# Autodesk Inventor assembly: Почти готово
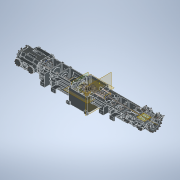
[picture p0: Inventor's stored thumbnail of the model, 180x180]
Saved by Autodesk Inventor 2021 (Build 250183000, 183)
## iProperties
Created: 2020-12-08
Part Number: Почти готово
Document SubType Name: Assembly
Designer: Тимоха
Author: Тимоха
## Documents named in this file (41)
- C:\Users\Тимоха\Desktop\КР Компрессор\compressor\Почти готово.iam
- C:\Users\Тимоха\Desktop\КР Компрессор\compressor\Картер.ipt
- C:\Users\Тимоха\Documents\Inventor\Content Center Files\R2021\ru-RU\Nut GOST 15524-70\Гайка M24-6H ГОСТ 15524-70.ipt
- C:\Users\Тимоха\Documents\Inventor\Content Center Files\R2021\ru-RU\GOST 11371-78  A\Шайба 27 ГОСТ 11371-78.ipt
- C:\Users\Тимоха\Desktop\КР Компрессор\compressor\Почти готово_CPY.iam
- C:\Users\Тимоха\Desktop\КР Компрессор\compressor\Вал.ipt
- C:\Users\Тимоха\Desktop\КР Компрессор\compressor\Нижняя часть коренного подшипника.ipt
- C:\Users\Тимоха\Desktop\КР Компрессор\compressor\Крышка коренного подшипника1.ipt
- C:\Users\Тимоха\Documents\Inventor\Content Center Files\R2021\ru-RU\Stud GOST 22038-76\Шпилька M24-6g×110 ГОСТ 22038-76.ipt
- C:\Users\Тимоха\Desktop\КР Компрессор\compressor\Под шатун.ipt
- C:\Users\Тимоха\Desktop\КР Компрессор\compressor\Шатун.ipt
- C:\Users\Тимоха\Desktop\КР Компрессор\compressor\Крышка стенки картера верх.ipt
- C:\Users\Тимоха\Desktop\КР Компрессор\compressor\Крышка стенки картера низ.ipt
- C:\Users\Тимоха\Desktop\КР Компрессор\compressor\Балка.ipt
- C:\Users\Тимоха\Documents\Inventor\Content Center Files\R2021\ru-RU\Bolt GOST R 50274-92\Болт M8-6g×16-F ГОСТ Р 50274-92.ipt
- C:\Users\Тимоха\Documents\Inventor\Content Center Files\R2021\ru-RU\Bolt GOST R 50274-92\Болт M8-6g×20-F ГОСТ Р 50274-92.ipt
- C:\Users\Тимоха\Desktop\КР Компрессор\compressor\Крышка картера 1.ipt
- C:\Users\Тимоха\Desktop\КР Компрессор\compressor\Крышка картера 2.ipt
- C:\Users\Тимоха\Desktop\КР Компрессор\compressor\Крышка картера 3.ipt
- C:\Users\Тимоха\Desktop\КР Компрессор\compressor\Крышка картера 4.ipt
- C:\Users\Тимоха\Desktop\КР Компрессор\compressor\Стяжка.ipt
- C:\Users\Тимоха\Documents\Inventor\Content Center Files\R2021\ru-RU\Nut GOST ISO 4034-2014\ГайкаM14ГОСТ ISO 4034-2014.ipt
- C:\Users\Тимоха\Desktop\КР Компрессор\compressor\Под стяжку.ipt
- C:\Users\Тимоха\Desktop\КР Компрессор\compressor\Под стяжку_MIR.ipt
- C:\Users\Тимоха\Desktop\КР Компрессор\compressor\Стяжка_MIR.ipt
- C:\Users\Тимоха\Desktop\КР Компрессор\compressor\Под стяжку_MIR1.ipt
- C:\Users\Тимоха\Desktop\КР Компрессор\compressor\Под стяжку_MIR_MIR.ipt
- C:\Users\Тимоха\Desktop\КР Компрессор\compressor\Корпус дросселя.ipt
- C:\Users\Тимоха\Desktop\КР Компрессор\compressor\Корпус сальника 1.ipt
- C:\Users\Тимоха\Desktop\КР Компрессор\compressor\Корпус сальника 2.ipt
- C:\Users\Тимоха\Desktop\КР Компрессор\compressor\Корпус сальника 3.ipt
- C:\Users\Тимоха\Desktop\КР Компрессор\compressor\Корпус сальника 4.ipt
- C:\Users\Тимоха\Desktop\КР Компрессор\compressor\Корпус сальника0.ipt
- C:\Users\Тимоха\Desktop\КР Компрессор\compressor\Крышка сальников.ipt
- C:\Users\Тимоха\Desktop\КР Компрессор\compressor\В сальник.ipt
- C:\Users\Тимоха\Desktop\КР Компрессор\compressor\Дроссельное кольцо.ipt
- C:\Users\Тимоха\Desktop\КР Компрессор\compressor\Кольцо сальника 1.ipt
- C:\Users\Тимоха\Desktop\КР Компрессор\compressor\Кольцо сальника 2.ipt
- C:\Users\Тимоха\Desktop\КР Компрессор\compressor\Кольцо сальника.ipt
- C:\Users\Тимоха\Desktop\КР Компрессор\compressor\Пружина дросселя.ipt
- C:\Users\Тимоха\Desktop\КР Компрессор\compressor\Пружина сальника.ipt
## Components (186 placed, 40 different names)
1. Картер:1 — Жесткий:406, Жесткий:407, Жесткий:410, Жесткий:411, Жесткий:412, Жесткий:421, Жесткий:422, Жесткий:423, Жесткий:428, Жесткий:429, Жесткий:431, Жесткий:433, Жесткий:434, Заподлицо:1, Заподлицо:2, Заподлицо:3, Заподлицо:4, Заподлицо:5, Заподлицо:6, Заподлицо:7, Заподлицо:8, Заподлицо:9, Жесткий:483, Жесткий:484, Заподлицо:14, Заподлицо:15, Заподлицо:16
2. Вал:1 — Цилиндрический:3, Жесткий:426, Совмещение:1, Жесткий:430, С поворотом:4
3. Нижняя часть коренного подшипника:1 — Жесткий:406, Цилиндрический:3, Жесткий:408
4. Нижняя часть коренного подшипника:2 — Жесткий:407, Жесткий:409
5. Нижняя часть коренного подшипника:3 — Жесткий:409
6. Нижняя часть коренного подшипника:4 — Жесткий:408
7. Крышка коренного подшипника1:1 — Жесткий:410
8. Крышка коренного подшипника1:2 — Жесткий:411, Совмещение:1
9. Шпилька ГОСТ 22038-76 M24-6g×110:1 — Жесткий:412, Жесткий:413, Жесткий:414
10. Гайка ГОСТ 15524-70 M24:54 — Жесткий:414
11. Шайба  ГОСТ 11371-78 28:22 — Жесткий:413
12. Шпилька ГОСТ 22038-76 M24-6g×110:2 — Жесткий:421
13. Гайка ГОСТ 15524-70 M24:55
14. Шайба  ГОСТ 11371-78 28:23
15. Шпилька ГОСТ 22038-76 M24-6g×110:3 — Жесткий:423
16. Гайка ГОСТ 15524-70 M24:56
17. Шайба  ГОСТ 11371-78 28:24
18. Шпилька ГОСТ 22038-76 M24-6g×110:4 — Жесткий:422
19. Гайка ГОСТ 15524-70 M24:57
20. Шайба  ГОСТ 11371-78 28:25
21. Под шатун:1 — Жесткий:425
22. Под шатун:2 — Жесткий:425, Жесткий:430
23. Под шатун:3 — Жесткий:426, Жесткий:427
24. Под шатун:4 — Жесткий:427, Цилиндрический:5
25. Почти готово_CPY:1 [sub-assembly] — Жесткий:429, С поворотом:5
26. Почти готово_CPY:2 [sub-assembly] — Жесткий:428, С поворотом:2, Заподлицо:7, Жесткий:546
27. Шатун:2 — Цилиндрический:5, С поворотом:2
28. Крышка стенки картера верх:1 — Жесткий:432, Жесткий:435, Жесткий:436, Жесткий:437, Жесткий:438, Жесткий:439, Жесткий:440, Жесткий:442, Жесткий:443, Жесткий:444, Жесткий:445, Жесткий:446, Жесткий:452, Жесткий:453, Жесткий:454, Жесткий:455, Жесткий:456, Жесткий:457, Жесткий:458
29. Крышка стенки картера низ:1 — Жесткий:431, Жесткий:432, Жесткий:447, Жесткий:448, Жесткий:449, Жесткий:450, Жесткий:451
30. Балка:1 — Жесткий:433
31. Балка:2 — Жесткий:434
32. Болт ГОСТ Р 50274-92 M8-6g×20-F:1 — Жесткий:435
33. Болт ГОСТ Р 50274-92 M8-6g×16-F:1 — Жесткий:439
34. Болт ГОСТ Р 50274-92 M8-6g×16-F:2 — Жесткий:436
35. Болт ГОСТ Р 50274-92 M8-6g×16-F:3 — Жесткий:440
36. Болт ГОСТ Р 50274-92 M8-6g×16-F:5 — Жесткий:438
37. Болт ГОСТ Р 50274-92 M8-6g×16-F:6 — Жесткий:442
38. Болт ГОСТ Р 50274-92 M8-6g×16-F:7 — Жесткий:437
39. Болт ГОСТ Р 50274-92 M8-6g×20-F:2 — Жесткий:443
40. Болт ГОСТ Р 50274-92 M8-6g×16-F:8 — Жесткий:446
41. Болт ГОСТ Р 50274-92 M8-6g×16-F:9 — Жесткий:444
42. Болт ГОСТ Р 50274-92 M8-6g×16-F:10 — Жесткий:450
43. Болт ГОСТ Р 50274-92 M8-6g×16-F:11 — Жесткий:451
44. Болт ГОСТ Р 50274-92 M8-6g×16-F:12 — Жесткий:445
45. Болт ГОСТ Р 50274-92 M8-6g×16-F:13 — Жесткий:447
46. Болт ГОСТ Р 50274-92 M8-6g×16-F:14 — Жесткий:449
47. Болт ГОСТ Р 50274-92 M8-6g×20-F:3 — Жесткий:452
48. Болт ГОСТ Р 50274-92 M8-6g×16-F:19 — Жесткий:448
49. Крышка картера 1:1 — Заподлицо:1, Заподлицо:2, Жесткий:459, Жесткий:460, Жесткий:461, Заподлицо:10, Жесткий:470, Жесткий:471, Жесткий:472, Жесткий:473, Жесткий:474, Жесткий:475, Жесткий:476
50. Крышка картера 2:1 — Заподлицо:3, Заподлицо:4, Жесткий:462, Жесткий:463, Жесткий:464, С поворотом:3, Жесткий:465, Жесткий:466, Жесткий:467, Заподлицо:11, Заподлицо:12
51. Крышка картера 3:1 — Заподлицо:5, Заподлицо:6, Жесткий:468, Жесткий:469, Заподлицо:13
52. Крышка картера 4:1 — Заподлицо:8, Заподлицо:9, Жесткий:477, Жесткий:478, Жесткий:479, Жесткий:480, Жесткий:481, Жесткий:482
53. Болт ГОСТ Р 50274-92 M8-6g×20-F:4 — Жесткий:453
54. Болт ГОСТ Р 50274-92 M8-6g×20-F:12 — Жесткий:471
55. Болт ГОСТ Р 50274-92 M8-6g×20-F:13 — Жесткий:473
56. Болт ГОСТ Р 50274-92 M8-6g×20-F:19 — Жесткий:468
57. Болт ГОСТ Р 50274-92 M8-6g×20-F:20 — Жесткий:469
58. Болт ГОСТ Р 50274-92 M8-6g×20-F:21 — Жесткий:460
59. Болт ГОСТ Р 50274-92 M8-6g×20-F:26 — Жесткий:454
60. Болт ГОСТ Р 50274-92 M8-6g×20-F:27 — Жесткий:463
61. Болт ГОСТ Р 50274-92 M8-6g×20-F:28 — Жесткий:462
62. Болт ГОСТ Р 50274-92 M8-6g×20-F:29 — Жесткий:458
63. Болт ГОСТ Р 50274-92 M8-6g×20-F:30 — Жесткий:465
64. Болт ГОСТ Р 50274-92 M8-6g×20-F:31 — Жесткий:466
65. Болт ГОСТ Р 50274-92 M8-6g×20-F:32 — Жесткий:467
66. Болт ГОСТ Р 50274-92 M8-6g×20-F:33 — Жесткий:455
67. Болт ГОСТ Р 50274-92 M8-6g×20-F:34 — Жесткий:456
68. Болт ГОСТ Р 50274-92 M8-6g×20-F:35 — Жесткий:457
69. Болт ГОСТ Р 50274-92 M8-6g×20-F:36 — Жесткий:461
70. Болт ГОСТ Р 50274-92 M8-6g×20-F:37 — Жесткий:459
71. Болт ГОСТ Р 50274-92 M8-6g×20-F:38 — Жесткий:464
72. Болт ГОСТ Р 50274-92 M8-6g×20-F:39 — С поворотом:3
73. Болт ГОСТ Р 50274-92 M8-6g×20-F:40 — Жесткий:470
74. Болт ГОСТ Р 50274-92 M8-6g×20-F:41 — Жесткий:472
75. Болт ГОСТ Р 50274-92 M8-6g×20-F:42 — Жесткий:474
76. Болт ГОСТ Р 50274-92 M8-6g×20-F:43 — Жесткий:475
77. Болт ГОСТ Р 50274-92 M8-6g×20-F:45 — Жесткий:476
78. Болт ГОСТ Р 50274-92 M8-6g×20-F:47
79. Болт ГОСТ Р 50274-92 M8-6g×20-F:48
80. Болт ГОСТ Р 50274-92 M8-6g×20-F:49
81. Болт ГОСТ Р 50274-92 M8-6g×20-F:50
82. Болт ГОСТ Р 50274-92 M8-6g×20-F:51
83. Болт ГОСТ Р 50274-92 M8-6g×20-F:52
84. Болт ГОСТ Р 50274-92 M8-6g×20-F:53
85. Болт ГОСТ Р 50274-92 M8-6g×20-F:54
86. Болт ГОСТ Р 50274-92 M8-6g×20-F:55
87. Болт ГОСТ Р 50274-92 M8-6g×20-F:56
88. Болт ГОСТ Р 50274-92 M8-6g×20-F:57
89. Болт ГОСТ Р 50274-92 M8-6g×20-F:58
90. Болт ГОСТ Р 50274-92 M8-6g×20-F:59
91. Болт ГОСТ Р 50274-92 M8-6g×20-F:60
92. Болт ГОСТ Р 50274-92 M8-6g×20-F:61
93. Болт ГОСТ Р 50274-92 M8-6g×20-F:62
94. Болт ГОСТ Р 50274-92 M8-6g×20-F:63
95. Болт ГОСТ Р 50274-92 M8-6g×20-F:64
96. Болт ГОСТ Р 50274-92 M8-6g×20-F:65
97. Болт ГОСТ Р 50274-92 M8-6g×20-F:66
98. Болт ГОСТ Р 50274-92 M8-6g×20-F:67
99. Болт ГОСТ Р 50274-92 M8-6g×20-F:68
100. Болт ГОСТ Р 50274-92 M8-6g×20-F:69
101. Болт ГОСТ Р 50274-92 M8-6g×20-F:70
102. Болт ГОСТ Р 50274-92 M8-6g×20-F:71
103. Болт ГОСТ Р 50274-92 M8-6g×20-F:72
104. Болт ГОСТ Р 50274-92 M8-6g×20-F:73
105. Болт ГОСТ Р 50274-92 M8-6g×20-F:74
106. Болт ГОСТ Р 50274-92 M8-6g×20-F:75
107. Болт ГОСТ Р 50274-92 M8-6g×20-F:76
108. Болт ГОСТ Р 50274-92 M8-6g×20-F:77
109. Болт ГОСТ Р 50274-92 M8-6g×20-F:78
110. Болт ГОСТ Р 50274-92 M8-6g×20-F:79
111. Болт ГОСТ Р 50274-92 M8-6g×20-F:80
112. Болт ГОСТ Р 50274-92 M8-6g×20-F:81
113. Болт ГОСТ Р 50274-92 M8-6g×20-F:82
114. Болт ГОСТ Р 50274-92 M8-6g×20-F:83
115. Болт ГОСТ Р 50274-92 M8-6g×20-F:84
116. Болт ГОСТ Р 50274-92 M8-6g×20-F:85
117. Болт ГОСТ Р 50274-92 M8-6g×20-F:86
118. Болт ГОСТ Р 50274-92 M8-6g×20-F:87 — Жесткий:477
119. Болт ГОСТ Р 50274-92 M8-6g×20-F:88 — Жесткий:478
120. Болт ГОСТ Р 50274-92 M8-6g×20-F:89 — Жесткий:480
121. Болт ГОСТ Р 50274-92 M8-6g×20-F:90 — Жесткий:481
122. Болт ГОСТ Р 50274-92 M8-6g×20-F:91 — Жесткий:479
123. Болт ГОСТ Р 50274-92 M8-6g×20-F:92 — Жесткий:482
124. Стяжка:1 — Жесткий:483
125. Гайка ГОСТ ISO 4034-2014 (M14):1 — Жесткий:485
126. Стяжка:2 — Жесткий:484
127. Под стяжку:1 — Заподлицо:14, Заподлицо:15, Жесткий:485, Жесткий:486
128. Гайка ГОСТ ISO 4034-2014 (M14):2 — Жесткий:486
129. Гайка ГОСТ ISO 4034-2014 (M14):3 — Жесткий:487
130. Под стяжку_MIR:1 — Жесткий:487, Жесткий:488
131. Гайка ГОСТ ISO 4034-2014 (M14):4 — Жесткий:488
132. Стяжка_MIR:1
133. Гайка ГОСТ ISO 4034-2014 (M14):5 — Жесткий:489
134. Стяжка_MIR:2
135. Под стяжку_MIR1:1 — Жесткий:489, Жесткий:490
136. Гайка ГОСТ ISO 4034-2014 (M14):6 — Жесткий:490
137. Гайка ГОСТ ISO 4034-2014 (M14):7 — Жесткий:491
138. Под стяжку_MIR_MIR:1 — Жесткий:491, Жесткий:492
139. Гайка ГОСТ ISO 4034-2014 (M14):8 — Жесткий:492
140. Шатун:3 — С поворотом:4, С поворотом:5
141. Корпус дросселя:2
142. Корпус сальника 1:2
143. Корпус сальника 2:2
144. Корпус сальника 3:2
145. Корпус сальника 4:2
146. Корпус сальника0:2
147. Крышка сальников:2 — Жесткий:546
148. В сальник:2
149. Дроссельное кольцо:1
150. Кольцо сальника 1:1
151. Кольцо сальника 2:1
152. Кольцо сальника:1
153. Пружина дросселя:1
154. Пружина сальника:1
155. Пружина сальника:2
156. Пружина сальника:3
157. Кольцо сальника:2
158. Пружина сальника:4
159. Кольцо сальника:3
160. Пружина сальника:5
161. Кольцо сальника:4
162. Пружина сальника:6
163. Кольцо сальника 1:2
164. Кольцо сальника 2:2
165. Кольцо сальника:5
166. Пружина сальника:7
167. Пружина сальника:8
168. Пружина сальника:9
169. Кольцо сальника:6
170. Пружина сальника:10
171. Кольцо сальника:7
172. Пружина сальника:11
173. Кольцо сальника:8
174. Пружина сальника:12
175. Кольцо сальника:9
176. Пружина сальника:13
177. Кольцо сальника:10
178. Пружина сальника:14
179. Кольцо сальника:11
180. Пружина сальника:15
181. Кольцо сальника:12
182. Пружина сальника:16
183. Кольцо сальника:13
184. Пружина сальника:17
185. Кольцо сальника:14
186. Пружина сальника:18
## Relationships (154: WeldJoint 131, Flush 16, RevoluteJoint 4, CylindricalJoint 2, Mate 1)
- Жесткий:406 [WeldJoint]: Картер:1 ↔ Нижняя часть коренного подшипника:1
- Жесткий:407 [WeldJoint]: Картер:1 ↔ Нижняя часть коренного подшипника:2
- Цилиндрический:3 [CylindricalJoint]: Вал:1 ↔ Нижняя часть коренного подшипника:1
- Жесткий:408 [WeldJoint]: Нижняя часть коренного подшипника:1 ↔ Нижняя часть коренного подшипника:4
- Жесткий:409 [WeldJoint]: Нижняя часть коренного подшипника:2 ↔ Нижняя часть коренного подшипника:3
- Жесткий:410 [WeldJoint]: Картер:1 ↔ Крышка коренного подшипника1:1
- Жесткий:411 [WeldJoint]: Картер:1 ↔ Крышка коренного подшипника1:2
- Жесткий:412 [WeldJoint]: Картер:1 ↔ Шпилька ГОСТ 22038-76 M24-6g×110:1
- Жесткий:413 [WeldJoint] (-35 mm): Шпилька ГОСТ 22038-76 M24-6g×110:1 ↔ Шайба  ГОСТ 11371-78 28:22
- Жесткий:414 [WeldJoint] (-5.75 mm): Шпилька ГОСТ 22038-76 M24-6g×110:1 ↔ Гайка ГОСТ 15524-70 M24:54
- [WeldJoint] (-35 mm): Шпилька ГОСТ 22038-76 M24-6g×110:2 ↔ Шайба  ГОСТ 11371-78 28:23
- [WeldJoint] (-5.75 mm): Шпилька ГОСТ 22038-76 M24-6g×110:2 ↔ Гайка ГОСТ 15524-70 M24:55
- [WeldJoint] (-35 mm): Шпилька ГОСТ 22038-76 M24-6g×110:3 ↔ Шайба  ГОСТ 11371-78 28:24
- [WeldJoint] (-5.75 mm): Шпилька ГОСТ 22038-76 M24-6g×110:3 ↔ Гайка ГОСТ 15524-70 M24:56
- [WeldJoint] (-35 mm): Шпилька ГОСТ 22038-76 M24-6g×110:4 ↔ Шайба  ГОСТ 11371-78 28:25
- [WeldJoint] (-5.75 mm): Шпилька ГОСТ 22038-76 M24-6g×110:4 ↔ Гайка ГОСТ 15524-70 M24:57
- Жесткий:421 [WeldJoint]: Картер:1 ↔ Шпилька ГОСТ 22038-76 M24-6g×110:2
- Жесткий:422 [WeldJoint]: Картер:1 ↔ Шпилька ГОСТ 22038-76 M24-6g×110:4
- Жесткий:423 [WeldJoint]: Картер:1 ↔ Шпилька ГОСТ 22038-76 M24-6g×110:3
- Жесткий:425 [WeldJoint]: Под шатун:1 ↔ Под шатун:2
- Жесткий:426 [WeldJoint]: Вал:1 ↔ Под шатун:3
- Жесткий:427 [WeldJoint]: Под шатун:3 ↔ Под шатун:4
- Жесткий:428 [WeldJoint]: Картер:1 ↔ Почти готово_CPY:2
- Жесткий:429 [WeldJoint]: Картер:1 ↔ Почти готово_CPY:1
- Цилиндрический:5 [CylindricalJoint]: Под шатун:4 ↔ Шатун:2
- С поворотом:2 [RevoluteJoint]: Почти готово_CPY:2 ↔ Шатун:2
- Совмещение:1 [Mate] (5 mm): Вал:1 ↔ Крышка коренного подшипника1:2
- Жесткий:430 [WeldJoint]: Вал:1 ↔ Под шатун:2
- Жесткий:431 [WeldJoint]: Картер:1 ↔ Крышка стенки картера низ:1
- Жесткий:432 [WeldJoint]: Крышка стенки картера верх:1 ↔ Крышка стенки картера низ:1
- Жесткий:433 [WeldJoint]: Картер:1 ↔ Балка:1
- Жесткий:434 [WeldJoint]: Картер:1 ↔ Балка:2
- Жесткий:435 [WeldJoint]: Крышка стенки картера верх:1 ↔ Болт ГОСТ Р 50274-92 M8-6g×20-F:1
- Жесткий:436 [WeldJoint]: Крышка стенки картера верх:1 ↔ Болт ГОСТ Р 50274-92 M8-6g×16-F:2
- Жесткий:437 [WeldJoint]: Крышка стенки картера верх:1 ↔ Болт ГОСТ Р 50274-92 M8-6g×16-F:7
- Жесткий:438 [WeldJoint]: Крышка стенки картера верх:1 ↔ Болт ГОСТ Р 50274-92 M8-6g×16-F:5
- Жесткий:439 [WeldJoint]: Крышка стенки картера верх:1 ↔ Болт ГОСТ Р 50274-92 M8-6g×16-F:1
- Жесткий:440 [WeldJoint]: Крышка стенки картера верх:1 ↔ Болт ГОСТ Р 50274-92 M8-6g×16-F:3
- Жесткий:442 [WeldJoint]: Крышка стенки картера верх:1 ↔ Болт ГОСТ Р 50274-92 M8-6g×16-F:6
- Жесткий:443 [WeldJoint]: Крышка стенки картера верх:1 ↔ Болт ГОСТ Р 50274-92 M8-6g×20-F:2
- Жесткий:444 [WeldJoint]: Крышка стенки картера верх:1 ↔ Болт ГОСТ Р 50274-92 M8-6g×16-F:9
- Жесткий:445 [WeldJoint]: Крышка стенки картера верх:1 ↔ Болт ГОСТ Р 50274-92 M8-6g×16-F:12
- Жесткий:446 [WeldJoint]: Крышка стенки картера верх:1 ↔ Болт ГОСТ Р 50274-92 M8-6g×16-F:8
- Жесткий:447 [WeldJoint]: Крышка стенки картера низ:1 ↔ Болт ГОСТ Р 50274-92 M8-6g×16-F:13
- Жесткий:448 [WeldJoint]: Крышка стенки картера низ:1 ↔ Болт ГОСТ Р 50274-92 M8-6g×16-F:19
- Жесткий:449 [WeldJoint]: Крышка стенки картера низ:1 ↔ Болт ГОСТ Р 50274-92 M8-6g×16-F:14
- Жесткий:450 [WeldJoint]: Крышка стенки картера низ:1 ↔ Болт ГОСТ Р 50274-92 M8-6g×16-F:10
- Жесткий:451 [WeldJoint]: Крышка стенки картера низ:1 ↔ Болт ГОСТ Р 50274-92 M8-6g×16-F:11
- Жесткий:452 [WeldJoint]: Крышка стенки картера верх:1 ↔ Болт ГОСТ Р 50274-92 M8-6g×20-F:3
- Заподлицо:1 [Flush]: Картер:1 ↔ Крышка картера 1:1
- Заподлицо:2 [Flush]: Картер:1 ↔ Крышка картера 1:1
- Заподлицо:3 [Flush]: Картер:1 ↔ Крышка картера 2:1
- Заподлицо:4 [Flush]: Картер:1 ↔ Крышка картера 2:1
- Заподлицо:5 [Flush]: Картер:1 ↔ Крышка картера 3:1
- Заподлицо:6 [Flush]: Картер:1 ↔ Крышка картера 3:1
- Заподлицо:7 [Flush]: Картер:1 ↔ Почти готово_CPY:2
- Заподлицо:8 [Flush]: Картер:1 ↔ Крышка картера 4:1
- Заподлицо:9 [Flush]: Картер:1 ↔ Крышка картера 4:1
- Жесткий:453 [WeldJoint]: Крышка стенки картера верх:1 ↔ Болт ГОСТ Р 50274-92 M8-6g×20-F:4
- Жесткий:454 [WeldJoint]: Крышка стенки картера верх:1 ↔ Болт ГОСТ Р 50274-92 M8-6g×20-F:26
- Жесткий:455 [WeldJoint]: Крышка стенки картера верх:1 ↔ Болт ГОСТ Р 50274-92 M8-6g×20-F:33
- Жесткий:456 [WeldJoint]: Крышка стенки картера верх:1 ↔ Болт ГОСТ Р 50274-92 M8-6g×20-F:34
- Жесткий:457 [WeldJoint]: Крышка стенки картера верх:1 ↔ Болт ГОСТ Р 50274-92 M8-6g×20-F:35
- Жесткий:458 [WeldJoint]: Крышка стенки картера верх:1 ↔ Болт ГОСТ Р 50274-92 M8-6g×20-F:29
- Жесткий:459 [WeldJoint]: Крышка картера 1:1 ↔ Болт ГОСТ Р 50274-92 M8-6g×20-F:37
- Жесткий:460 [WeldJoint]: Крышка картера 1:1 ↔ Болт ГОСТ Р 50274-92 M8-6g×20-F:21
- Жесткий:461 [WeldJoint]: Крышка картера 1:1 ↔ Болт ГОСТ Р 50274-92 M8-6g×20-F:36
- Жесткий:462 [WeldJoint]: Крышка картера 2:1 ↔ Болт ГОСТ Р 50274-92 M8-6g×20-F:28
- Жесткий:463 [WeldJoint]: Крышка картера 2:1 ↔ Болт ГОСТ Р 50274-92 M8-6g×20-F:27
- Жесткий:464 [WeldJoint]: Крышка картера 2:1 ↔ Болт ГОСТ Р 50274-92 M8-6g×20-F:38
- С поворотом:3 [RevoluteJoint]: Крышка картера 2:1 ↔ Болт ГОСТ Р 50274-92 M8-6g×20-F:39
- Жесткий:465 [WeldJoint]: Крышка картера 2:1 ↔ Болт ГОСТ Р 50274-92 M8-6g×20-F:30
- Жесткий:466 [WeldJoint]: Крышка картера 2:1 ↔ Болт ГОСТ Р 50274-92 M8-6g×20-F:31
- Жесткий:467 [WeldJoint]: Крышка картера 2:1 ↔ Болт ГОСТ Р 50274-92 M8-6g×20-F:32
- Жесткий:468 [WeldJoint]: Крышка картера 3:1 ↔ Болт ГОСТ Р 50274-92 M8-6g×20-F:19
- Жесткий:469 [WeldJoint]: Крышка картера 3:1 ↔ Болт ГОСТ Р 50274-92 M8-6g×20-F:20
- Заподлицо:10 [Flush] (8 mm): Крышка картера 1:1
- Заподлицо:11 [Flush] (-326.9 mm): Крышка картера 2:1
- Заподлицо:12 [Flush] (8 mm): Крышка картера 2:1
- Заподлицо:13 [Flush] (-66.5 mm): Крышка картера 3:1
- Жесткий:470 [WeldJoint]: Крышка картера 1:1 ↔ Болт ГОСТ Р 50274-92 M8-6g×20-F:40
- Жесткий:471 [WeldJoint]: Крышка картера 1:1 ↔ Болт ГОСТ Р 50274-92 M8-6g×20-F:12
- Жесткий:472 [WeldJoint]: Крышка картера 1:1 ↔ Болт ГОСТ Р 50274-92 M8-6g×20-F:41
- Жесткий:473 [WeldJoint]: Крышка картера 1:1 ↔ Болт ГОСТ Р 50274-92 M8-6g×20-F:13
- Жесткий:474 [WeldJoint]: Крышка картера 1:1 ↔ Болт ГОСТ Р 50274-92 M8-6g×20-F:42
- Жесткий:475 [WeldJoint]: Крышка картера 1:1 ↔ Болт ГОСТ Р 50274-92 M8-6g×20-F:43
- Жесткий:476 [WeldJoint]: Крышка картера 1:1 ↔ Болт ГОСТ Р 50274-92 M8-6g×20-F:45
- Жесткий:477 [WeldJoint]: Крышка картера 4:1 ↔ Болт ГОСТ Р 50274-92 M8-6g×20-F:87
- Жесткий:478 [WeldJoint]: Крышка картера 4:1 ↔ Болт ГОСТ Р 50274-92 M8-6g×20-F:88
- Жесткий:479 [WeldJoint]: Крышка картера 4:1 ↔ Болт ГОСТ Р 50274-92 M8-6g×20-F:91
- Жесткий:480 [WeldJoint]: Крышка картера 4:1 ↔ Болт ГОСТ Р 50274-92 M8-6g×20-F:89
- Жесткий:481 [WeldJoint]: Крышка картера 4:1 ↔ Болт ГОСТ Р 50274-92 M8-6g×20-F:90
- Жесткий:482 [WeldJoint]: Крышка картера 4:1 ↔ Болт ГОСТ Р 50274-92 M8-6g×20-F:92
- Жесткий:483 [WeldJoint] (-40 mm): Картер:1 ↔ Стяжка:1
- Жесткий:484 [WeldJoint] (40 mm): Картер:1 ↔ Стяжка:2
- Заподлицо:14 [Flush]: Картер:1 ↔ Под стяжку:1
- Заподлицо:15 [Flush]: Картер:1 ↔ Под стяжку:1
- Жесткий:485 [WeldJoint]: Гайка ГОСТ ISO 4034-2014 (M14):1 ↔ Под стяжку:1
- Жесткий:486 [WeldJoint]: Под стяжку:1 ↔ Гайка ГОСТ ISO 4034-2014 (M14):2
- Жесткий:487 [WeldJoint]: Гайка ГОСТ ISO 4034-2014 (M14):3 ↔ Под стяжку_MIR:1
- Жесткий:488 [WeldJoint]: Под стяжку_MIR:1 ↔ Гайка ГОСТ ISO 4034-2014 (M14):4
- Заподлицо:16 [Flush] (-465 mm): Картер:1
- Жесткий:489 [WeldJoint]: Гайка ГОСТ ISO 4034-2014 (M14):5 ↔ Под стяжку_MIR1:1
- Жесткий:490 [WeldJoint]: Под стяжку_MIR1:1 ↔ Гайка ГОСТ ISO 4034-2014 (M14):6
- Жесткий:491 [WeldJoint]: Гайка ГОСТ ISO 4034-2014 (M14):7 ↔ Под стяжку_MIR_MIR:1
- Жесткий:492 [WeldJoint]: Под стяжку_MIR_MIR:1 ↔ Гайка ГОСТ ISO 4034-2014 (M14):8
- С поворотом:4 [RevoluteJoint]: Вал:1 ↔ Шатун:3
- С поворотом:5 [RevoluteJoint]: Почти готово_CPY:1 ↔ Шатун:3
- [WeldJoint]: Корпус дросселя:2 ↔ Корпус сальника0:2
- [WeldJoint]: Корпус сальника 1:2 ↔ Корпус сальника0:2
- [WeldJoint]: Корпус сальника 1:2 ↔ Корпус сальника 2:2
- [WeldJoint]: Корпус сальника 2:2 ↔ Корпус сальника 3:2
- [WeldJoint]: Корпус сальника 3:2 ↔ Корпус сальника 4:2
- [WeldJoint]: Корпус сальника 4:2 ↔ В сальник:2
- [WeldJoint]: Крышка сальников:2 ↔ В сальник:2
- [WeldJoint]: Кольцо сальника:1 ↔ Пружина сальника:2
- [WeldJoint]: Кольцо сальника 2:1 ↔ Пружина сальника:3
- [WeldJoint]: Кольцо сальника 1:1 ↔ Пружина сальника:1
- [WeldJoint]: Дроссельное кольцо:1 ↔ Пружина дросселя:1
- [WeldJoint]: Кольцо сальника:2 ↔ Пружина сальника:4
- [WeldJoint]: Кольцо сальника:3 ↔ Пружина сальника:5
- [WeldJoint]: Кольцо сальника:4 ↔ Пружина сальника:6
- [WeldJoint]: Кольцо сальника:2 ↔ Кольцо сальника:3
- [WeldJoint]: Кольцо сальника:3 ↔ Кольцо сальника:4
- [WeldJoint]: Кольцо сальника 1:1 ↔ Кольцо сальника 2:1
- [WeldJoint]: Кольцо сальника 1:1 ↔ Кольцо сальника:1
- [WeldJoint]: Кольцо сальника:5 ↔ Пружина сальника:8
- [WeldJoint]: Кольцо сальника 2:2 ↔ Пружина сальника:9
- [WeldJoint]: Кольцо сальника 1:2 ↔ Пружина сальника:7
- [WeldJoint]: Кольцо сальника 1:2 ↔ Кольцо сальника 2:2
- [WeldJoint]: Кольцо сальника 1:2 ↔ Кольцо сальника:5
- [WeldJoint]: Кольцо сальника:6 ↔ Пружина сальника:10
- [WeldJoint]: Кольцо сальника:7 ↔ Пружина сальника:11
- [WeldJoint]: Кольцо сальника:8 ↔ Пружина сальника:12
- [WeldJoint]: Кольцо сальника:6 ↔ Кольцо сальника:7
- [WeldJoint]: Кольцо сальника:7 ↔ Кольцо сальника:8
- [WeldJoint]: Кольцо сальника:9 ↔ Пружина сальника:13
- [WeldJoint]: Кольцо сальника:10 ↔ Пружина сальника:14
- [WeldJoint]: Кольцо сальника:11 ↔ Пружина сальника:15
- [WeldJoint]: Кольцо сальника:9 ↔ Кольцо сальника:10
- [WeldJoint]: Кольцо сальника:10 ↔ Кольцо сальника:11
- [WeldJoint]: Кольцо сальника:12 ↔ Пружина сальника:16
- [WeldJoint]: Кольцо сальника:13 ↔ Пружина сальника:17
- [WeldJoint]: Кольцо сальника:14 ↔ Пружина сальника:18
- [WeldJoint]: Кольцо сальника:12 ↔ Кольцо сальника:13
- [WeldJoint]: Кольцо сальника:13 ↔ Кольцо сальника:14
- [WeldJoint]: Корпус дросселя:2 ↔ Дроссельное кольцо:1
- [WeldJoint]: Корпус сальника0:2 ↔ Кольцо сальника:4
- [WeldJoint]: Корпус сальника 1:2 ↔ Кольцо сальника:14
- [WeldJoint]: Корпус сальника 2:2 ↔ Кольцо сальника:8
- [WeldJoint]: Корпус сальника 3:2 ↔ Кольцо сальника:11
- [WeldJoint]: Корпус сальника 4:2 ↔ Кольцо сальника:1
- [WeldJoint]: Крышка сальников:2 ↔ Кольцо сальника:5
- Жесткий:546 [WeldJoint] (3 mm): Почти готово_CPY:2 ↔ Крышка сальников:2
## Named parameters: d482_d480 = -35 mm, d483_d481 = -5.75 mm, d484_d480 = -35 mm, d485_d481 = -5.75 mm, d486_d480 = -35 mm, d487_d481 = -5.75 mm, d28_d11_d7 = 0 mm, d29_d12_d7 = 0 mm, d30_d13_d7 = 0 mm, d31_d14 = 0 mm, d32_d15 = 0 mm, d33_d11_d7 = 0 mm, d34_d12_d7 = 0 mm, d35_d13_d7 = 0 mm, d36_d14 = 0 mm, d37_d15 = 0 mm, d11_d7 = 0 mm, d12_d7 = 0 mm, d13_d7 = 0 mm, d18_d7 = 0 mm, d19_d8 = 0 mm, d20_d9 = 0 mm, d21_d16 = 0 mm, d22_d17 = 0 mm, d23_d11_d7 = 0 mm, d24_d12_d7 = 0 mm, d25_d13_d7 = 0 mm, d26_d14 = 0 mm, d27_d15 = 0 mm, d645_d599 = 0 mm, d646_d600 = 0 mm, d647_d601 = 0 mm, d648_d602 = 0 mm, d649_d603 = 0 mm, d650_d604 = 0 mm, d651_d605 = 0 mm
